# Autodesk Inventor assembly: wahacz_zewn_szkic
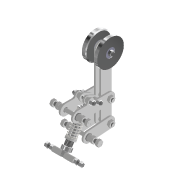
[picture p0: Inventor's stored thumbnail of the model, 180x180]
Saved by Autodesk Inventor 2020.3 (Build 243373000, 373)
## iProperties
Created: 2021-10-24
Part Number: wahacz_zewn_szkic
Document SubType Name: Assembly
Designer: patry
Author: patry
## Documents named in this file (22)
- C:\Users\patry\Desktop\Semestr 7\Inzynierka\Projekt inventor\Ariadna_inzynierka\Workspaces\Obszar roboczy\Obszar roboczy\Naped\Zawieszenie_v3\wahacz_zewn_szkic.iam
- C:\Users\patry\Desktop\Semestr 7\Inzynierka\Projekt inventor\Ariadna_inzynierka\Workspaces\Obszar roboczy\Obszar roboczy\Naped\Zawieszenie_v3\ramie_1_wahacza.ipt
- C:\Users\patry\Desktop\Semestr 7\Inzynierka\Projekt inventor\Ariadna_inzynierka\Workspaces\Obszar roboczy\Obszar roboczy\Naped\Zawieszenie_v3\ramie_2_wahacza.ipt
- C:\Users\patry\Desktop\Semestr 7\Inzynierka\Projekt inventor\Ariadna_inzynierka\Workspaces\Obszar roboczy\Obszar roboczy\Naped\Zawieszenie_v3\tuleja_TUF106040.ipt
- C:\Users\patry\Desktop\Semestr 7\Inzynierka\Projekt inventor\Ariadna_inzynierka\Workspaces\Obszar roboczy\Obszar roboczy\Naped\Sruby\M6_nut_5mm.ipt
- C:\Users\patry\Desktop\Semestr 7\Inzynierka\Projekt inventor\Ariadna_inzynierka\Workspaces\Obszar roboczy\Obszar roboczy\Naped\Sruby\M5_nut_5mm.ipt
- C:\Users\patry\Desktop\Semestr 7\Inzynierka\Projekt inventor\Ariadna_inzynierka\Workspaces\Obszar roboczy\Obszar roboczy\Naped\Sruby\M5_70_shaft.ipt
- C:\Users\patry\Desktop\Semestr 7\Inzynierka\Projekt inventor\Ariadna_inzynierka\Workspaces\Obszar roboczy\Obszar roboczy\Naped\Sruby\M3_16_shaft.ipt
- C:\Users\patry\Desktop\Semestr 7\Inzynierka\Projekt inventor\Ariadna_inzynierka\Workspaces\Obszar roboczy\Obszar roboczy\Naped\Sruby\M3_nut_2,5mm.ipt
- C:\Users\patry\Desktop\Semestr 7\Inzynierka\Projekt inventor\Ariadna_inzynierka\Workspaces\Obszar roboczy\Obszar roboczy\Naped\Zawieszenie_v3\wspornik_amortyzatora.ipt
- C:\Users\patry\Desktop\Semestr 7\Inzynierka\Projekt inventor\Ariadna_inzynierka\Workspaces\Obszar roboczy\Obszar roboczy\Naped\Sruby\M6_40_shaft.ipt
- C:\Users\patry\Desktop\Semestr 7\Inzynierka\Projekt inventor\Ariadna_inzynierka\Workspaces\Obszar roboczy\Obszar roboczy\Naped\Sruby\tuleja_M6_M10_7.ipt
- C:\Users\patry\Desktop\Semestr 7\Inzynierka\Projekt inventor\Ariadna_inzynierka\Workspaces\Obszar roboczy\Obszar roboczy\Naped\Sruby\M6_1,25_pad.ipt
- C:\Users\patry\Desktop\Semestr 7\Inzynierka\Projekt inventor\Ariadna_inzynierka\Workspaces\Obszar roboczy\Obszar roboczy\Naped\Sruby\M6_70_shaft.ipt
- C:\Users\patry\Desktop\Semestr 7\Inzynierka\Projekt inventor\Ariadna_inzynierka\Workspaces\Obszar roboczy\Obszar roboczy\Naped\Sruby\M5_40_shaft.ipt
- M5_shaft.ipt
- C:\Users\patry\Desktop\Semestr 7\Inzynierka\Projekt inventor\Ariadna_inzynierka\Workspaces\Obszar roboczy\Obszar roboczy\Naped\Sruby\tuleja_M5_M9_4,5.ipt
- C:\Users\patry\Desktop\Semestr 7\Inzynierka\Projekt inventor\Ariadna_inzynierka\Workspaces\Obszar roboczy\Obszar roboczy\Naped\Zawieszenie_v3\glowny_wahacz_zewn.ipt
- C:\Users\patry\Desktop\Semestr 7\Inzynierka\Projekt inventor\Ariadna_inzynierka\Workspaces\Obszar roboczy\Obszar roboczy\Naped\Zawieszenie_v3\independent_wheel_pair.iam
- C:\Users\patry\Desktop\Semestr 7\Inzynierka\Projekt inventor\Ariadna_inzynierka\Workspaces\Obszar roboczy\Obszar roboczy\Naped\Sruby\tuleja_M6_M10_6.ipt
- C:\Users\patry\Desktop\Semestr 7\Inzynierka\Projekt inventor\Ariadna_inzynierka\Workspaces\Obszar roboczy\Obszar roboczy\Naped\Sruby\tuleja_M5_M9_17.5.ipt
- C:\Users\patry\Desktop\Semestr 7\Inzynierka\Projekt inventor\Ariadna_inzynierka\Workspaces\Obszar roboczy\Obszar roboczy\Naped\Amortyzator\elemenet_sprężysty_zaw.iam
## Components (69 placed, 20 different names)
1. ramie_1_wahacza:1 — Zestawiające:7, Zestawiające:8, Kątowe:4, Zestawiające:108, Zestawiające:109, Zestawiające:110, Równoległe:6, Zestawiające:114, Zestawiające:158, Równoległe:11, Zestawiające:159, Równoległe:12, Zestawiające:161, Zestawiające:163, Zestawiające:175, Zestawiające:179, Zestawiające:203, Zestawiające:204, Równoległe:14, Kątowe:27
2. ramie_2_wahacza:1 — Zestawiające:1, Zestawiające:2, Kątowe:1, Zestawiające:118, Zestawiające:206, Zestawiające:207, Kątowe:10
3. tuleja_TUF106040:1 — Zestawiające:1, Zestawiające:2, Kątowe:1, Zestawiające:93, Zestawiające:200
4. tuleja_TUF106040:2 — Zestawiające:205, Zestawiające:206, Zestawiające:207, Zestawiające:238
5. tuleja_TUF106040:3 — Zestawiające:202, Zestawiające:203, Zestawiające:204
6. tuleja_TUF106040:4 — Zestawiające:7, Zestawiające:8, Kątowe:4, Zestawiające:111, Zestawiające:132
7. tuleja_TUF106040:5 — Zestawiające:89, Zestawiające:201, Zestawiające:240
8. tuleja_TUF106040:6 — Zestawiające:88, Zestawiające:90, Zestawiające:189, Zestawiające:198
9. ramie_2_wahacza:2 — Równoległe:7, Zestawiające:120, Zestawiające:209, Zestawiające:210
10. tuleja_TUF106040:7 — Zestawiające:93, Zestawiające:112, Zestawiające:140
11. tuleja_TUF106040:8 — Zestawiające:208, Zestawiające:209, Zestawiające:210, Zestawiające:236
12. M6_nut_5mm:2 — Zestawiające:113, Zestawiające:114, Kątowe:24, Kątowe:25
13. M5_nut_5mm:1 — Zestawiające:84, Zestawiające:86, Równoległe:9, Równoległe:10, Zestawiające:242, Równoległe:16, Kątowe:31
14. M5_70_shaft:1 — Zestawiające:84, Zestawiające:85, Zestawiające:143, Równoległe:8, Zestawiające:241, Zestawiające:243, Zestawiające:245, Zestawiające:247, Zestawiające:252, Równoległe:16
15. ramie_1_wahacza:3 — Zestawiające:88, Zestawiające:89, Zestawiające:90, Zestawiające:116, Zestawiające:165, Zestawiające:167, Zestawiające:173, Zestawiające:177, Zestawiające:201, Zestawiające:224, Równoległe:13, Kątowe:11
16. M5_nut_5mm:2 — Zestawiające:85, Zestawiające:86, Zestawiające:244, Kątowe:28, Kątowe:29
17. M3_16_shaft:1 — Zestawiające:97, Równoległe:5, Zestawiające:98, Zestawiające:100, Zestawiające:250
18. M3_nut_2,5mm:1 — Zestawiające:98, Zestawiające:99
19. M3_nut_2,5mm:2 — Zestawiające:100, Zestawiające:101
20. wspornik_amortyzatora:1 — Zestawiające:94, Zestawiające:95, Zestawiające:96, Równoległe:5, Zestawiające:99, Zestawiające:108, Zestawiające:109, Zestawiające:110, Zestawiające:251
21. wspornik_amortyzatora:2 — Zestawiające:94, Zestawiające:95, Zestawiające:96, Zestawiające:97, Zestawiające:101
22. M6_40_shaft:1 — Zestawiające:111, Równoległe:6, Zestawiające:113, Zestawiające:115, Zestawiające:121, Zestawiające:127, Zestawiające:131, Zestawiające:182, Zestawiające:186, Zestawiające:189
23. M6_40_shaft:2 — Zestawiające:112, Równoległe:7, Zestawiające:117, Zestawiające:119, Zestawiające:123, Zestawiające:135, Zestawiające:139, Zestawiające:180, Zestawiające:185
24. M6_nut_5mm:11 — Zestawiające:115, Zestawiające:116, Kątowe:19, Kątowe:20, Kątowe:21
25. M6_nut_5mm:12 — Zestawiające:117, Zestawiające:118, Kątowe:20
26. M6_nut_5mm:13 — Zestawiające:119, Zestawiające:120, Kątowe:23, Kątowe:24
27. tuleja_M6_M10_7:1 — Zestawiające:121, Zestawiające:196
28. tuleja_M6_M10_7:2 — Zestawiające:123, Zestawiające:181
29. M6_1,25_pad:1 — Zestawiające:125, Zestawiające:126, Zestawiające:127, Zestawiające:197
30. M6_1,25_pad:2 — Zestawiające:125, Zestawiające:126, Zestawiające:198
31. M6_1,25_pad:3 — Zestawiające:131, Zestawiające:132
32. M6_1,25_pad:4 — Zestawiające:194
33. M6_1,25_pad:5 — Zestawiające:135, Zestawiające:199
34. M6_1,25_pad:6 — Zestawiające:200
35. M6_1,25_pad:7 — Zestawiające:139, Zestawiające:140
36. M6_1,25_pad:8 — Zestawiające:195
37. M6_70_shaft:1 — Zestawiające:143, Zestawiające:149, Zestawiające:205, Zestawiające:208, Zestawiające:225, Zestawiające:227, Zestawiające:235, Zestawiające:237
38. M6_70_shaft:2 — Równoległe:8, Zestawiające:144, Zestawiające:145, Zestawiające:202, Zestawiające:229, Zestawiające:231, Zestawiające:233, Zestawiające:239
39. M6_nut_5mm:14 — Zestawiające:144, Zestawiające:146, Zestawiające:230, Kątowe:15
40. M6_nut_5mm:15 — Zestawiające:145, Zestawiające:146, Równoległe:9, Zestawiające:232, Kątowe:17, Kątowe:18
41. M6_nut_5mm:16 — Zestawiające:148, Zestawiające:149, Zestawiające:228, Kątowe:12, Kątowe:28
42. M6_nut_5mm:17 — Zestawiające:148, Równoległe:10, Zestawiające:226, Kątowe:14, Kątowe:18, Kątowe:19
43. M5_shaft:1 — Zestawiające:158, Równoległe:11, Zestawiające:162, Zestawiające:164, Zestawiające:172, Zestawiające:174
44. M5_shaft:2 — Zestawiające:159, Równoległe:12, Zestawiające:160, Zestawiające:166, Zestawiające:176, Zestawiające:178, Zestawiające:224
45. M5_nut_5mm:3 — Zestawiające:160, Zestawiające:161, Kątowe:25, Kątowe:26
46. M5_nut_5mm:4 — Zestawiające:162, Zestawiające:163, Kątowe:26
47. M5_nut_5mm:5 — Zestawiające:164, Zestawiające:165, Kątowe:22
48. M5_nut_5mm:6 — Zestawiające:166, Zestawiające:167, Kątowe:21, Kątowe:22
49. tuleja_M5_M9_4,5:1 — Zestawiające:172, Zestawiające:173
50. tuleja_M5_M9_4,5:2 — Zestawiające:174, Zestawiające:175
51. tuleja_M5_M9_4,5:3 — Zestawiające:176, Zestawiające:177
52. tuleja_M5_M9_4,5:4 — Zestawiające:178, Zestawiające:179
53. lacznik_zewn:1 — Zestawiające:180, Zestawiające:181, Zestawiające:182, Zestawiające:196, Zestawiające:197, Zestawiające:199, Zestawiające:249, Równoległe:15, Kątowe:10
54. lacznik_zewn:2 — Zestawiające:185, Zestawiające:186, Zestawiające:194, Zestawiające:195, Zestawiające:221, Zestawiające:222, Zestawiające:223
55. independent_wheel_pair:1 [sub-assembly] — Zestawiające:221, Zestawiające:222, Zestawiające:249
56. tuleja_M6_M10_7:3 — Zestawiające:223
57. tuleja_M6_M10_6:1 — Zestawiające:233, Zestawiające:234
58. M6_nut_5mm:18 — Zestawiające:225, Zestawiające:226, Kątowe:13, Kątowe:14
59. M6_nut_5mm:19 — Zestawiające:227, Zestawiające:228, Kątowe:12, Kątowe:13, Kątowe:23, Kątowe:27
60. M6_nut_5mm:20 — Zestawiające:229, Zestawiające:230, Zestawiające:234, Kątowe:15, Kątowe:16
61. M6_nut_5mm:21 — Zestawiające:231, Zestawiające:232, Kątowe:16, Kątowe:17
62. tuleja_M6_M10_6:2 — Zestawiające:235, Zestawiające:236
63. tuleja_M6_M10_6:3 — Zestawiające:237, Zestawiające:238
64. tuleja_M6_M10_6:4 — Zestawiające:239, Zestawiające:240
65. M5_nut_5mm:7 — Zestawiające:241, Zestawiające:242, Kątowe:30, Kątowe:31
66. M5_nut_5mm:8 — Zestawiające:243, Zestawiające:244, Zestawiające:246, Kątowe:29, Kątowe:30
67. tuleja_M5_M9_17.5:1 — Zestawiające:247, Zestawiające:256
68. tuleja_M5_M9_17.5:2 — Zestawiające:245, Zestawiające:246, Zestawiające:253
69. elemenet_sprężysty_zaw:1 [sub-assembly] — Zestawiające:250, Zestawiające:251, Zestawiające:252, Zestawiające:253, Kątowe:11, Zestawiające:256
## Relationships (169: Mate 132, Angle 25, Flush 12)
- Zestawiające:1 [Mate]: ramie_2_wahacza:1 ↔ tuleja_TUF106040:1
- Zestawiające:2 [Mate]: ramie_2_wahacza:1 ↔ tuleja_TUF106040:1
- Kątowe:1 [Angle] (0 deg): ramie_2_wahacza:1 ↔ tuleja_TUF106040:1
- Zestawiające:7 [Mate]: ramie_1_wahacza:1 ↔ tuleja_TUF106040:4
- Zestawiające:8 [Mate]: ramie_1_wahacza:1 ↔ tuleja_TUF106040:4
- Kątowe:4 [Angle] (0 deg): ramie_1_wahacza:1 ↔ tuleja_TUF106040:4
- [Mate]: ramie_2_wahacza:2 ↔ tuleja_TUF106040:7
- [Mate]: ramie_2_wahacza:2 ↔ tuleja_TUF106040:7
- [Angle] (0 deg): ramie_2_wahacza:2 ↔ tuleja_TUF106040:7
- Zestawiające:84 [Mate]: M5_nut_5mm:1 ↔ M5_70_shaft:1
- Zestawiające:85 [Mate]: M5_70_shaft:1 ↔ M5_nut_5mm:2
- Zestawiające:86 [Mate] (60 mm): M5_nut_5mm:1 ↔ M5_nut_5mm:2
- Zestawiające:88 [Mate]: tuleja_TUF106040:6 ↔ ramie_1_wahacza:3
- Zestawiające:89 [Mate]: tuleja_TUF106040:5 ↔ ramie_1_wahacza:3
- Zestawiające:90 [Mate]: tuleja_TUF106040:6 ↔ ramie_1_wahacza:3
- Zestawiające:93 [Mate]: tuleja_TUF106040:1 ↔ tuleja_TUF106040:7
- Zestawiające:94 [Mate]: wspornik_amortyzatora:1 ↔ wspornik_amortyzatora:2
- Zestawiające:95 [Mate]: wspornik_amortyzatora:1 ↔ wspornik_amortyzatora:2
- Zestawiające:96 [Mate] (5 mm): wspornik_amortyzatora:1 ↔ wspornik_amortyzatora:2
- Zestawiające:97 [Mate]: M3_16_shaft:1 ↔ wspornik_amortyzatora:2
- Równoległe:5 [Flush] (-2.5 mm): M3_16_shaft:1 ↔ wspornik_amortyzatora:1
- Zestawiające:98 [Mate]: M3_16_shaft:1 ↔ M3_nut_2,5mm:1
- Zestawiające:99 [Mate]: M3_nut_2,5mm:1 ↔ wspornik_amortyzatora:1
- Zestawiające:100 [Mate]: M3_16_shaft:1 ↔ M3_nut_2,5mm:2
- Zestawiające:101 [Mate]: M3_nut_2,5mm:2 ↔ wspornik_amortyzatora:2
- Zestawiające:108 [Mate]: ramie_1_wahacza:1 ↔ wspornik_amortyzatora:1
- Zestawiające:109 [Mate]: ramie_1_wahacza:1 ↔ wspornik_amortyzatora:1
- Zestawiające:110 [Mate] (4.5 mm): ramie_1_wahacza:1 ↔ wspornik_amortyzatora:1
- Zestawiające:111 [Mate]: tuleja_TUF106040:4 ↔ M6_40_shaft:1
- Równoległe:6 [Flush] (7 mm): ramie_1_wahacza:1 ↔ M6_40_shaft:1
- Zestawiające:112 [Mate]: tuleja_TUF106040:7 ↔ M6_40_shaft:2
- Równoległe:7 [Flush] (7 mm): ramie_2_wahacza:2 ↔ M6_40_shaft:2
- Zestawiające:113 [Mate]: M6_nut_5mm:2 ↔ M6_40_shaft:1
- Zestawiające:114 [Mate]: ramie_1_wahacza:1 ↔ M6_nut_5mm:2
- Zestawiające:115 [Mate]: M6_40_shaft:1 ↔ M6_nut_5mm:11
- Zestawiające:116 [Mate]: ramie_1_wahacza:3 ↔ M6_nut_5mm:11
- Zestawiające:117 [Mate]: M6_40_shaft:2 ↔ M6_nut_5mm:12
- Zestawiające:118 [Mate]: ramie_2_wahacza:1 ↔ M6_nut_5mm:12
- Zestawiające:119 [Mate]: M6_40_shaft:2 ↔ M6_nut_5mm:13
- Zestawiające:120 [Mate]: ramie_2_wahacza:2 ↔ M6_nut_5mm:13
- Zestawiające:121 [Mate]: M6_40_shaft:1 ↔ tuleja_M6_M10_7:1
- Zestawiające:123 [Mate]: M6_40_shaft:2 ↔ tuleja_M6_M10_7:2
- Zestawiające:125 [Mate]: M6_1,25_pad:1 ↔ M6_1,25_pad:2
- Zestawiające:126 [Mate]: M6_1,25_pad:1 ↔ M6_1,25_pad:2
- Zestawiające:127 [Mate]: M6_40_shaft:1 ↔ M6_1,25_pad:1
- [Mate]: M6_1,25_pad:3 ↔ M6_1,25_pad:4
- [Mate]: M6_1,25_pad:3 ↔ M6_1,25_pad:4
- Zestawiające:131 [Mate]: M6_40_shaft:1 ↔ M6_1,25_pad:3
- Zestawiające:132 [Mate]: tuleja_TUF106040:4 ↔ M6_1,25_pad:3
- [Mate]: M6_1,25_pad:5 ↔ M6_1,25_pad:6
- [Mate]: M6_1,25_pad:5 ↔ M6_1,25_pad:6
- Zestawiające:135 [Mate]: M6_40_shaft:2 ↔ M6_1,25_pad:5
- [Mate]: M6_1,25_pad:7 ↔ M6_1,25_pad:8
- [Mate]: M6_1,25_pad:7 ↔ M6_1,25_pad:8
- Zestawiające:139 [Mate]: M6_40_shaft:2 ↔ M6_1,25_pad:7
- Zestawiające:140 [Mate]: tuleja_TUF106040:7 ↔ M6_1,25_pad:7
- Zestawiające:143 [Mate]: M5_70_shaft:1 ↔ M6_70_shaft:1
- Równoległe:8 [Flush]: M5_70_shaft:1 ↔ M6_70_shaft:2
- Zestawiające:144 [Mate]: M6_70_shaft:2 ↔ M6_nut_5mm:14
- Zestawiające:145 [Mate]: M6_70_shaft:2 ↔ M6_nut_5mm:15
- Zestawiające:146 [Mate] (60 mm): M6_nut_5mm:14 ↔ M6_nut_5mm:15
- Równoległe:9 [Flush]: M5_nut_5mm:1 ↔ M6_nut_5mm:15
- [Mate] (60 mm): M6_nut_5mm:16 ↔ M6_nut_5mm:17
- Zestawiające:148 [Mate]: M6_nut_5mm:16 ↔ M6_nut_5mm:17
- Zestawiające:149 [Mate]: M6_70_shaft:1 ↔ M6_nut_5mm:16
- Równoległe:10 [Flush]: M5_nut_5mm:1 ↔ M6_nut_5mm:17
- Zestawiające:158 [Mate]: ramie_1_wahacza:1 ↔ M5_shaft:1
- Równoległe:11 [Flush] (7 mm): ramie_1_wahacza:1 ↔ M5_shaft:1
- Zestawiające:159 [Mate]: ramie_1_wahacza:1 ↔ M5_shaft:2
- Równoległe:12 [Flush] (7 mm): ramie_1_wahacza:1 ↔ M5_shaft:2
- Zestawiające:160 [Mate]: M5_shaft:2 ↔ M5_nut_5mm:3
- Zestawiające:161 [Mate]: ramie_1_wahacza:1 ↔ M5_nut_5mm:3
- Zestawiające:162 [Mate]: M5_shaft:1 ↔ M5_nut_5mm:4
- Zestawiające:163 [Mate]: ramie_1_wahacza:1 ↔ M5_nut_5mm:4
- Zestawiające:164 [Mate]: M5_shaft:1 ↔ M5_nut_5mm:5
- Zestawiające:165 [Mate]: ramie_1_wahacza:3 ↔ M5_nut_5mm:5
- Zestawiające:166 [Mate]: M5_shaft:2 ↔ M5_nut_5mm:6
- Zestawiające:167 [Mate]: ramie_1_wahacza:3 ↔ M5_nut_5mm:6
- Zestawiające:172 [Mate]: M5_shaft:1 ↔ tuleja_M5_M9_4,5:1
- Zestawiające:173 [Mate]: ramie_1_wahacza:3 ↔ tuleja_M5_M9_4,5:1
- Zestawiające:174 [Mate]: M5_shaft:1 ↔ tuleja_M5_M9_4,5:2
- Zestawiające:175 [Mate]: ramie_1_wahacza:1 ↔ tuleja_M5_M9_4,5:2
- Zestawiające:176 [Mate]: M5_shaft:2 ↔ tuleja_M5_M9_4,5:3
- Zestawiające:177 [Mate]: ramie_1_wahacza:3 ↔ tuleja_M5_M9_4,5:3
- Zestawiające:178 [Mate]: M5_shaft:2 ↔ tuleja_M5_M9_4,5:4
- Zestawiające:179 [Mate]: ramie_1_wahacza:1 ↔ tuleja_M5_M9_4,5:4
- Zestawiające:180 [Mate]: M6_40_shaft:2 ↔ lacznik_zewn:1
- Zestawiające:181 [Mate]: tuleja_M6_M10_7:2 ↔ lacznik_zewn:1
- Zestawiające:182 [Mate]: M6_40_shaft:1 ↔ lacznik_zewn:1
- Zestawiające:185 [Mate]: M6_40_shaft:2 ↔ lacznik_zewn:2
- Zestawiające:186 [Mate]: M6_40_shaft:1 ↔ lacznik_zewn:2
- Zestawiające:189 [Mate]: tuleja_TUF106040:6 ↔ M6_40_shaft:1
- Zestawiające:194 [Mate]: M6_1,25_pad:4 ↔ lacznik_zewn:2
- Zestawiające:195 [Mate]: M6_1,25_pad:8 ↔ lacznik_zewn:2
- Zestawiające:196 [Mate]: tuleja_M6_M10_7:1 ↔ lacznik_zewn:1
- Zestawiające:197 [Mate]: M6_1,25_pad:1 ↔ lacznik_zewn:1
- Zestawiające:198 [Mate]: tuleja_TUF106040:6 ↔ M6_1,25_pad:2
- Zestawiające:199 [Mate]: M6_1,25_pad:5 ↔ lacznik_zewn:1
- Zestawiające:200 [Mate]: tuleja_TUF106040:1 ↔ M6_1,25_pad:6
- Zestawiające:201 [Mate]: tuleja_TUF106040:5 ↔ ramie_1_wahacza:3
- Zestawiające:202 [Mate]: tuleja_TUF106040:3 ↔ M6_70_shaft:2
- Zestawiające:203 [Mate]: ramie_1_wahacza:1 ↔ tuleja_TUF106040:3
- Zestawiające:204 [Mate]: ramie_1_wahacza:1 ↔ tuleja_TUF106040:3
- Zestawiające:205 [Mate]: tuleja_TUF106040:2 ↔ M6_70_shaft:1
- Zestawiające:206 [Mate]: ramie_2_wahacza:1 ↔ tuleja_TUF106040:2
- Zestawiające:207 [Mate]: ramie_2_wahacza:1 ↔ tuleja_TUF106040:2
- Zestawiające:208 [Mate]: tuleja_TUF106040:8 ↔ M6_70_shaft:1
- Zestawiające:209 [Mate]: ramie_2_wahacza:2 ↔ tuleja_TUF106040:8
- Zestawiające:210 [Mate]: ramie_2_wahacza:2 ↔ tuleja_TUF106040:8
- [Mate]: independent_wheel_pair:1 ↔ tuleja_M6_M10_7:3
- Zestawiające:221 [Mate]: lacznik_zewn:2 ↔ independent_wheel_pair:1
- Zestawiające:222 [Mate]: lacznik_zewn:2 ↔ independent_wheel_pair:1
- Zestawiające:223 [Mate]: lacznik_zewn:2 ↔ tuleja_M6_M10_7:3
- Zestawiające:224 [Mate]: ramie_1_wahacza:3 ↔ M5_shaft:2
- Zestawiające:225 [Mate]: M6_70_shaft:1 ↔ M6_nut_5mm:18
- Zestawiające:226 [Mate] (5 mm): M6_nut_5mm:17 ↔ M6_nut_5mm:18
- Zestawiające:227 [Mate]: M6_70_shaft:1 ↔ M6_nut_5mm:19
- Zestawiające:228 [Mate] (5 mm): M6_nut_5mm:16 ↔ M6_nut_5mm:19
- Zestawiające:229 [Mate]: M6_70_shaft:2 ↔ M6_nut_5mm:20
- Zestawiające:230 [Mate] (5 mm): M6_nut_5mm:14 ↔ M6_nut_5mm:20
- Zestawiające:231 [Mate]: M6_70_shaft:2 ↔ M6_nut_5mm:21
- Zestawiające:232 [Mate] (5 mm): M6_nut_5mm:15 ↔ M6_nut_5mm:21
- Zestawiające:233 [Mate]: M6_70_shaft:2 ↔ tuleja_M6_M10_6:1
- Zestawiające:234 [Mate]: tuleja_M6_M10_6:1 ↔ M6_nut_5mm:20
- Zestawiające:235 [Mate]: M6_70_shaft:1 ↔ tuleja_M6_M10_6:2
- Zestawiające:236 [Mate]: tuleja_TUF106040:8 ↔ tuleja_M6_M10_6:2
- Zestawiające:237 [Mate]: M6_70_shaft:1 ↔ tuleja_M6_M10_6:3
- Zestawiające:238 [Mate]: tuleja_TUF106040:2 ↔ tuleja_M6_M10_6:3
- Zestawiające:239 [Mate]: M6_70_shaft:2 ↔ tuleja_M6_M10_6:4
- Zestawiające:240 [Mate]: tuleja_TUF106040:5 ↔ tuleja_M6_M10_6:4
- Zestawiające:241 [Mate]: M5_70_shaft:1 ↔ M5_nut_5mm:7
- Zestawiające:242 [Mate] (5 mm): M5_nut_5mm:1 ↔ M5_nut_5mm:7
- Zestawiające:243 [Mate]: M5_70_shaft:1 ↔ M5_nut_5mm:8
- Zestawiające:244 [Mate] (5 mm): M5_nut_5mm:2 ↔ M5_nut_5mm:8
- Zestawiające:245 [Mate]: M5_70_shaft:1 ↔ tuleja_M5_M9_17.5:2
- Zestawiające:246 [Mate]: M5_nut_5mm:8 ↔ tuleja_M5_M9_17.5:2
- Zestawiające:247 [Mate]: M5_70_shaft:1 ↔ tuleja_M5_M9_17.5:1
- Zestawiające:249 [Mate]: lacznik_zewn:1 ↔ independent_wheel_pair:1
- Równoległe:13 [Flush]: ramie_1_wahacza:3
- Równoległe:14 [Flush]: ramie_1_wahacza:1
- Równoległe:15 [Flush]: lacznik_zewn:1
- Kątowe:10 [Angle] (-85.65 deg): ramie_2_wahacza:1 ↔ lacznik_zewn:1
- Zestawiające:250 [Mate]: M3_16_shaft:1 ↔ elemenet_sprężysty_zaw:1
- Zestawiające:251 [Mate]: wspornik_amortyzatora:1 ↔ elemenet_sprężysty_zaw:1
- Zestawiające:252 [Mate]: M5_70_shaft:1 ↔ elemenet_sprężysty_zaw:1
- Równoległe:16 [Flush]: M5_nut_5mm:1 ↔ M5_70_shaft:1
- Zestawiające:253 [Mate]: tuleja_M5_M9_17.5:2 ↔ elemenet_sprężysty_zaw:1
- Kątowe:11 [Angle] (-31.81 deg): ramie_1_wahacza:3 ↔ elemenet_sprężysty_zaw:1
- Zestawiające:256 [Mate]: tuleja_M5_M9_17.5:1 ↔ elemenet_sprężysty_zaw:1
- Kątowe:12 [Angle] (0 deg): M6_nut_5mm:16 ↔ M6_nut_5mm:19
- Kątowe:13 [Angle] (0 deg): M6_nut_5mm:18 ↔ M6_nut_5mm:19
- Kątowe:14 [Angle] (0 deg): M6_nut_5mm:17 ↔ M6_nut_5mm:18
- Kątowe:15 [Angle] (0 deg): M6_nut_5mm:14 ↔ M6_nut_5mm:20
- Kątowe:16 [Angle] (0 deg): M6_nut_5mm:20 ↔ M6_nut_5mm:21
- Kątowe:17 [Angle] (0 deg): M6_nut_5mm:15 ↔ M6_nut_5mm:21
- Kątowe:18 [Angle] (0 deg): M6_nut_5mm:15 ↔ M6_nut_5mm:17
- Kątowe:19 [Angle] (0 deg): M6_nut_5mm:11 ↔ M6_nut_5mm:17
- Kątowe:20 [Angle] (0 deg): M6_nut_5mm:11 ↔ M6_nut_5mm:12
- Kątowe:21 [Angle] (0 deg): M6_nut_5mm:11 ↔ M5_nut_5mm:6
- Kątowe:22 [Angle] (0 deg): M5_nut_5mm:5 ↔ M5_nut_5mm:6
- Kątowe:23 [Angle] (0 deg): M6_nut_5mm:13 ↔ M6_nut_5mm:19
- Kątowe:24 [Angle] (0 deg): M6_nut_5mm:2 ↔ M6_nut_5mm:13
- Kątowe:25 [Angle] (0 deg): M6_nut_5mm:2 ↔ M5_nut_5mm:3
- Kątowe:26 [Angle] (0 deg): M5_nut_5mm:3 ↔ M5_nut_5mm:4
- Kątowe:27 [Angle] (0 deg): ramie_1_wahacza:1 ↔ M6_nut_5mm:19
- Kątowe:28 [Angle] (0 deg): M5_nut_5mm:2 ↔ M6_nut_5mm:16
- Kątowe:29 [Angle] (0 deg): M5_nut_5mm:2 ↔ M5_nut_5mm:8
- Kątowe:30 [Angle] (0 deg): M5_nut_5mm:7 ↔ M5_nut_5mm:8
- Kątowe:31 [Angle] (0 deg): M5_nut_5mm:1 ↔ M5_nut_5mm:7
## Named parameters: d41_d4 = 0 deg, d43_d0 = 0 mm, d44_d1 = 0 mm, d158_d154 = 0 mm, d159_d155 = 0 mm, d162_d154 = 0 mm, d163_d155 = 0 mm, d166_d154 = 0 mm, d167_d155 = 0 mm, d178_d176 = 60 mm
